# Autodesk Inventor assembly: Ascensor uvas + riel1
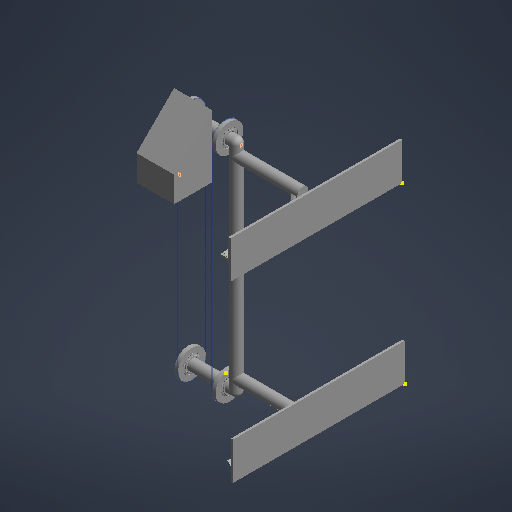
[picture p0: Inventor's stored thumbnail of the model, 512x512]
Saved by Autodesk Inventor 2026.2 (Build 302298010, 298A)
## iProperties
Part Number: Ascensor uvas + riel1
Document SubType Name: Assembly
Designer: diego
Author: diego
## Documents named in this file (13)
- C:\Users\agusb\Desktop\Monsters University\Universidad\semestre_3\Dis_grafico\proyecto\Ascensor uvas + riel1.iam
- C:\Users\agusb\Desktop\Monsters University\Universidad\semestre_3\Dis_grafico\proyecto\Union_Poleas.ipt
- C:\Users\agusb\Desktop\Monsters University\Universidad\semestre_3\Dis_grafico\proyecto\Rueda.ipt
- C:\Users\agusb\Desktop\Monsters University\Universidad\semestre_3\Dis_grafico\proyecto\ISO 4014 - M14 x 90 - ISO.ipt
- C:\Users\agusb\Desktop\Monsters University\Universidad\semestre_3\Dis_grafico\proyecto\ISO 4161 - M14(1).ipt
- C:\Users\agusb\Desktop\Monsters University\Universidad\semestre_3\Dis_grafico\proyecto\Riel superior.ipt
- C:\Users\agusb\Desktop\Monsters University\Universidad\semestre_3\Dis_grafico\proyecto\Riel Inferior.ipt
- C:\Users\agusb\Desktop\Monsters University\Universidad\semestre_3\Dis_grafico\proyecto\rodamiento\skf_bearing_t2ee_100_2.iam
- C:\Users\agusb\Desktop\Monsters University\Universidad\semestre_3\Dis_grafico\archivos\Proyecto\Cajon_ascensor_mejor.ipt
- C:\Users\agusb\Desktop\Monsters University\Universidad\semestre_3\Dis_grafico\proyecto\rodamiento\exterior_rodamiento.ipt
- C:\Users\agusb\Desktop\Monsters University\Universidad\semestre_3\Dis_grafico\proyecto\Ascensor uvas + riel1\Design Accelerator\Transmisión por cadena1.iam
- C:\Users\agusb\Desktop\Monsters University\Universidad\semestre_3\Dis_grafico\proyecto\Ascensor uvas + riel1\Design Accelerator\Transmisión por cadena2.iam
- C:\Users\agusb\Desktop\Monsters University\Universidad\semestre_3\Dis_grafico\archivos\Proyecto\pasador_cajon.ipt
## Components (21 placed, 11 different names)
1. Union_Poleas:1 — Coincidencia:1, Coincidencia:2, Coincidencia:3, Coincidencia:4, De rotación:2, Coincidencia:5, Coincidencia:6, Coincidencia:7, Coincidencia:8, De rotación:3, De rotación:4, Cilíndrica:1, Cilíndrica:2, Cilíndrica:3, Cilíndrica:4
2. Rueda:2 — De rotación:2, De rotación:4
3. ISO 4014 M14 x 90:1 — Coincidencia:1, Coincidencia:2
4. ISO 4161 M14:1 — Coincidencia:3, Coincidencia:4
5. ISO 4014 M14 x 90:2 — Coincidencia:5, Coincidencia:6
6. ISO 4161 M14:2 — Coincidencia:7, Coincidencia:8
7. Rueda:3 — De rotación:3
8. Riel superior:1
9. Riel Inferior:1
10. skf_bearing_t2ee_100_2:1 [sub-assembly] — Cilíndrica:2, De rotación:5
11. skf_bearing_t2ee_100_2:2 [sub-assembly] — Cilíndrica:3, De rotación:8
12. skf_bearing_t2ee_100_2:3 [sub-assembly] — Cilíndrica:1, De rotación:6
13. skf_bearing_t2ee_100_2:4 [sub-assembly] — Cilíndrica:4, De rotación:7
14. Cajon_ascensor_mejor:1 — De rotación:9
15. exterior_rodamiento:1 — De rotación:7
16. exterior_rodamiento:2 — De rotación:5
17. exterior_rodamiento:3 — De rotación:6
18. exterior_rodamiento:4 — De rotación:8
19. Transmisión por cadena:1 [sub-assembly] — Coincidencia:11
20. Transmisión por cadena:2 [sub-assembly] — Coincidencia:10
21. pasador_cajon:1 — Coincidencia:10, Coincidencia:11, De rotación:9
## Relationships (22: Mate 10, RevoluteJoint 8, CylindricalJoint 4)
- Coincidencia:1 [Mate]: Union_Poleas:1 ↔ ISO 4014 M14 x 90:1
- Coincidencia:2 [Mate]: Union_Poleas:1 ↔ ISO 4014 M14 x 90:1
- Coincidencia:3 [Mate]: Union_Poleas:1 ↔ ISO 4161 M14:1
- Coincidencia:4 [Mate]: Union_Poleas:1 ↔ ISO 4161 M14:1
- De rotación:2 [RevoluteJoint]: Union_Poleas:1 ↔ Rueda:2
- Coincidencia:5 [Mate]: Union_Poleas:1 ↔ ISO 4014 M14 x 90:2
- Coincidencia:6 [Mate]: Union_Poleas:1 ↔ ISO 4014 M14 x 90:2
- Coincidencia:7 [Mate]: Union_Poleas:1 ↔ ISO 4161 M14:2
- Coincidencia:8 [Mate]: Union_Poleas:1 ↔ ISO 4161 M14:2
- De rotación:3 [RevoluteJoint]: Union_Poleas:1 ↔ Rueda:3
- De rotación:4 [RevoluteJoint]: Union_Poleas:1 ↔ Rueda:2
- Cilíndrica:1 [CylindricalJoint]: Union_Poleas:1 ↔ skf_bearing_t2ee_100_2:3
- Cilíndrica:2 [CylindricalJoint]: Union_Poleas:1 ↔ skf_bearing_t2ee_100_2:1
- Cilíndrica:3 [CylindricalJoint]: Union_Poleas:1 ↔ skf_bearing_t2ee_100_2:2
- Cilíndrica:4 [CylindricalJoint]: Union_Poleas:1 ↔ skf_bearing_t2ee_100_2:4
- De rotación:5 [RevoluteJoint]: skf_bearing_t2ee_100_2:1 ↔ exterior_rodamiento:2
- De rotación:6 [RevoluteJoint]: skf_bearing_t2ee_100_2:3 ↔ exterior_rodamiento:3
- De rotación:7 [RevoluteJoint]: skf_bearing_t2ee_100_2:4 ↔ exterior_rodamiento:1
- De rotación:8 [RevoluteJoint]: skf_bearing_t2ee_100_2:2 ↔ exterior_rodamiento:4
- Coincidencia:10 [Mate]: Transmisión por cadena:2 ↔ pasador_cajon:1
- Coincidencia:11 [Mate]: Transmisión por cadena:1 ↔ pasador_cajon:1
- De rotación:9 [RevoluteJoint]: Cajon_ascensor_mejor:1 ↔ pasador_cajon:1
